# Autodesk Inventor assembly: Wheel Right
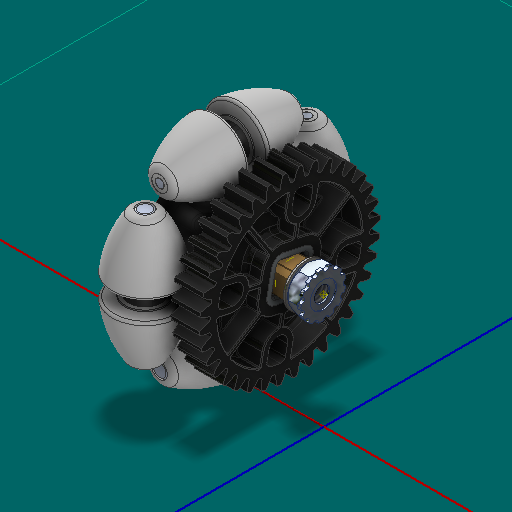
[picture p0: Inventor's stored thumbnail of the model, 512x512]
Saved by Autodesk Inventor 2025 (Build 290162000, 162)
## iProperties
Created: 2024-10-18
Part Number: Wheel Right
Document SubType Name: Assembly
Designer: Averey Ku
Author: averey
## Documents named in this file (7)
- C:\Users\avere\VEX\High Stakes\CAD\V2\Chassis\Drivebay Right\Wheel Right.iam
- C:\Users\avere\VEX\High Stakes\CAD\V2\Chassis\Drivebay Right\Half Cut HS 36T Gear, No Insert Right.ipt
- C:\Users\avere\VEX\High Stakes\CAD\V2\Chassis\Drivebay Right\HS Shaft Adapter Circle Right.ipt
- C:\Users\avere\VEX\High Stakes\CAD\V2\Chassis\Drivebay Right\Nut Keps Right2.ipt
- C:\Users\avere\VEX\High Stakes\CAD\ROBOPROS-CAD-Inventor\Motion\Spacers\Washer Steel\SWasher .375 OD x .015625.ipt
- C:\Users\avere\VEX\High Stakes\CAD\V2\Chassis\Drivebay Right\2.00 Omni AS, No Insert Right.ipt
- C:\Users\avere\VEX\High Stakes\CAD\ROBOPROS-CAD-Inventor\Motion\Spacers\Washer Steel.ipt
## Components (7 placed, 5 different names)
1. Half Cut HS 36T Gear, No Insert Right:1 — Angle:1, Insert:6
2. HS Shaft Adapter Circle Right:1 — Angle:1, Insert:4, Insert:1
3. Nut Keps Right2:1 — Mate:1, Insert:2
4. SWasher .375 OD x .015625:1 — Insert:4, Insert:5
5. 2.00 Omni AS, No Insert Right:1 — Insert:6, Insert:5
6. SWasher .375 OD x .015625:2 — Insert:2, Insert:3
7. HS Shaft Adapter Circle Right:2 — Insert:3, Insert:1
## Relationships (8: Insert 6, Angle 1, Mate 1)
- Angle:1 (0 deg): Half Cut HS 36T Gear, No Insert Right:1 ↔ HS Shaft Adapter Circle Right:1
- Mate:1: Nut Keps Right2:1
- Insert:4: HS Shaft Adapter Circle Right:1 ↔ SWasher .375 OD x .015625:1
- Insert:6: Half Cut HS 36T Gear, No Insert Right:1 ↔ 2.00 Omni AS, No Insert Right:1
- Insert:5: SWasher .375 OD x .015625:1 ↔ 2.00 Omni AS, No Insert Right:1
- Insert:2: Nut Keps Right2:1 ↔ SWasher .375 OD x .015625:2
- Insert:3: SWasher .375 OD x .015625:2 ↔ HS Shaft Adapter Circle Right:2
- Insert:1: HS Shaft Adapter Circle Right:1 ↔ HS Shaft Adapter Circle Right:2
